# Autodesk Inventor assembly: Whole-body-cuvette-30x30x120
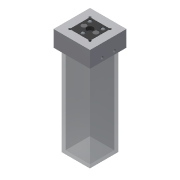
[picture p0: Inventor's stored thumbnail of the model, 180x180]
Saved by Autodesk Inventor 2019 (Build 230136000, 136)
## iProperties
Created: 2019-09-25
Part Number: Whole-body-cuvette-30x30x120
Document SubType Name: Assembly
Designer: voigt
Author: voigt
## Documents named in this file (4)
- J:\Microscope_Design\CAD_Files\mesoSPIM_design_V5.2\mesoSPIM\sample_handling\Whole-body-cuvettes\Whole-body-cuvette-30x30x120.iam
- J:\Microscope_Design\CAD_Files\mesoSPIM_design_V5.2\library\Portmann Instruments\UG-752-30x30x120mm.ipt
- J:\Microscope_Design\CAD_Files\mesoSPIM_design_V5.2\mesoSPIM\immersion_cuvette_mounts\Large-cuvette-mount-30mm-V1.ipt
- J:\Microscope_Design\CAD_Files\mesoSPIM_design_V5.2\library\Thorlabs\kinematic_bases\KBT25_top_steelballs_simplified.ipt
## Components (3 placed, 3 different names)
1. UG-752-30x30x120mm:1 — Mate:1, Flush:1, Mate:2, Mate:3, Mate:4, Mate:5
2. Large-cuvette-mount-30mm-V1:1 — Mate:3, Mate:4, Mate:5, Mate:6, Mate:7, Mate:8
3. KBT25_top_steelballs_simplified:1 — Mate:6, Mate:7, Mate:8
## Relationships (9: Mate 8, Flush 1)
- Mate:1: UG-752-30x30x120mm:1
- Flush:1 (-17.5 mm): UG-752-30x30x120mm:1
- Mate:2 (-17.5 mm): UG-752-30x30x120mm:1
- Mate:3: UG-752-30x30x120mm:1 ↔ Large-cuvette-mount-30mm-V1:1
- Mate:4: UG-752-30x30x120mm:1 ↔ Large-cuvette-mount-30mm-V1:1
- Mate:5: UG-752-30x30x120mm:1 ↔ Large-cuvette-mount-30mm-V1:1
- Mate:6: Large-cuvette-mount-30mm-V1:1 ↔ KBT25_top_steelballs_simplified:1
- Mate:7: Large-cuvette-mount-30mm-V1:1 ↔ KBT25_top_steelballs_simplified:1
- Mate:8: Large-cuvette-mount-30mm-V1:1 ↔ KBT25_top_steelballs_simplified:1
